# Autodesk Inventor assembly: RR-PCSS-2021-3M1
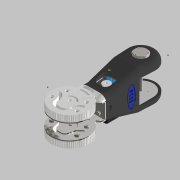
[picture p0: Inventor's stored thumbnail of the model, 180x180]
Saved by Autodesk Inventor 2021 (Build 250183000, 183)
## iProperties
Created: 2021-10-25
Part Number: RR-PCSS-2021-3M1
Document SubType Name: Assembly
Designer: marci
Mass: 2425.99 g
Surface Area: 3551.52 cm^2
Volume: 1267.26 cm^3
Density: 1.91436 g/cm^3
Author: marci
## Documents named in this file (25)
- C:\Users\marci\Desktop\Projekt ramienia\3M1D\RR-PCSS-2021-3M1.iam
- C:\Users\marci\Desktop\Projekt ramienia\3M1D\RR-PCSS-2021-3M1D.ipt
- C:\Users\marci\Desktop\Projekt ramienia\3M1D\RR-PCSS-2021-W3M1.1.ipt
- C:\Users\marci\Desktop\Projekt ramienia\3M1D\RR-PCSS-2021-MSK.ipt
- C:\Users\marci\Desktop\Projekt ramienia\3M1D\Nema 17 Reductor.ipt
- C:\Users\marci\Desktop\Projekt ramienia\3M1D\Pulley 8mm IGNIS.ipt
- C:\Users\marci\Desktop\Projekt ramienia\2M2\RR-PCSS-2021-W2M2MA.ipt
- C:\Users\marci\Desktop\Projekt ramienia\Nowy folder\pl-PL\ISO 4762(2)\ISO 4762 - M6 x 12ISO.ipt
- C:\Users\marci\Desktop\Projekt ramienia\Nowy folder\pl-PL\ISO 7089\ISO 7089 - 6 - 140 HV(1).ipt
- C:\Users\marci\Desktop\Projekt ramienia\Nowy folder\pl-PL\ISO 4035(2)\ISO 4035 - M6 - ISO.ipt
- C:\Users\marci\Desktop\Projekt ramienia\2M2\RR-PCSS-2021-2M2.ipt
- C:\Users\marci\Desktop\Projekt ramienia\Nowy folder\pl-PL\ANSI B18.3.1M(6)\ANSI B18.3.1M - M3x0,5 x 45(1).ipt
- C:\Users\marci\Desktop\Projekt ramienia\Nowy folder\pl-PL\ISO 7092\ISO 7092 - ST 3 - 140 HV.ipt
- C:\Users\marci\Desktop\Projekt ramienia\Nowy folder\pl-PL\ISO 4036(2)\ISO 4036 - M3(2).ipt
- C:\Users\marci\Desktop\Projekt ramienia\3M1D\Tapa 3M1C.ipt
- C:\Users\marci\Desktop\Projekt ramienia\3M1D\T3M1.iam
- C:\Users\marci\Desktop\Projekt ramienia\Nowy folder\pl-PL\ISO 4762(2)\ISO 4762 - M4 x 6ISO.ipt
- C:\Users\marci\Desktop\Projekt ramienia\Nowy folder\pl-PL\ISO 4762(2)\ISO 4762 - M3 x 25ISO.ipt
- C:\Users\marci\Desktop\Projekt ramienia\Nowy folder\pl-PL\ISO 4762(2)\ISO 4762 - M5 x 16ISO.ipt
- C:\Users\marci\Desktop\Projekt ramienia\Nowy folder\pl-PL\ISO 4762(2)\ISO 4762 - M3 x 6ISO.ipt
- C:\Users\marci\Desktop\Projekt ramienia\3M1D\8mm Bearing.ipt
- C:\Users\marci\Desktop\Projekt ramienia\Nowy folder\pl-PL\ISO 4161\ISO 4161 - M8(1).ipt
- C:\Users\marci\Desktop\Projekt ramienia\Nowy folder\pl-PL\ISO 4762(2)\ISO 4762 - M6 x 20ISO.ipt
- C:\Users\marci\Desktop\Projekt ramienia\Nowy folder\pl-PL\ISO 4161\ISO 4161 - M6(1).ipt
- C:\Users\marci\Desktop\Projekt ramienia\Nowy folder\pl-PL\AS 1111\AS 1111 - M8 x 120.ipt
## Components (59 placed, 24 different names)
1. RR-PCSS-2021-W3M1.1:1 — Wstawiające:1, Zestawiające:1, Równoległe:1, Zestawiające:2, Zestawiające:8, Zestawiające:9, Zestawiające:11, Zestawiające:12, Zestawiające:13, Zestawiające:14, Zestawiające:15, Zestawiające:16, Zestawiające:17, Zestawiające:18, Zestawiające:19, Zestawiające:21, Zestawiające:23, Zestawiające:25
2. RR-PCSS-2021-3M1D:1 — Wstawiające:1, Zestawiające:27, Zestawiające:28, Zestawiające:29, Zestawiające:30, Zestawiające:31, Zestawiające:33, Zestawiające:34, Zestawiające:35, Zestawiające:36, Zestawiające:37, Zestawiające:50, Zestawiające:51, Zestawiające:52, Wstawiające:11, Wstawiające:12
3. RR-PCSS-2021-MSK:1 — Zestawiające:1, Równoległe:1, Zestawiające:2, Wstawiające:2, Zestawiające:32, Zestawiające:39, Zestawiające:40, Zestawiające:41, Zestawiające:42, Zestawiające:43, Zestawiające:53, Zestawiające:54, Zestawiające:55, Zestawiające:56, Zestawiające:57, Zestawiające:58, Zestawiające:59, Zestawiające:60
4. Nema 17 Reductor:1 — Wstawiające:2, Wstawiające:3, Zestawiające:10
5. Pulley 8mm IGNIS:1 — Wstawiające:3
6. RR-PCSS-2021-W2M2MA:1 — Zestawiające:8, Zestawiające:9, Zestawiające:10, Zestawiające:20, Zestawiające:22, Zestawiające:24, Zestawiające:26, Wstawiające:8, Wstawiające:9, Zestawiające:80, Zestawiające:82, Zestawiające:84, Zestawiające:86, Zestawiające:96, Zestawiające:98, Zestawiające:100, Zestawiające:102
7. ISO 4762 M6 x 12:1 — Zestawiające:11, Zestawiające:12
8. ISO 7089 6:1 — Zestawiające:19, Zestawiające:20, Wstawiające:4
9. ISO 4035 M6:1 — Wstawiające:4
10. ISO 4762 M6 x 12:2 — Zestawiające:13, Zestawiające:14
11. ISO 4762 M6 x 12:3 — Zestawiające:15, Zestawiające:16
12. ISO 4762 M6 x 12:4 — Zestawiające:17, Zestawiające:18
13. ISO 7089 6:2 — Zestawiające:21, Zestawiające:22, Wstawiające:5
14. ISO 7089 6:3 — Zestawiające:23, Zestawiające:24, Wstawiające:6
15. ISO 7089 6:4 — Zestawiające:25, Zestawiające:26, Wstawiające:7
16. ISO 4035 M6:2 — Wstawiające:5
17. ISO 4035 M6:3 — Wstawiające:6
18. ISO 4035 M6:4 — Wstawiające:7
19. RR-PCSS-2021-2M2:1 — Wstawiające:9, Zestawiające:28, Zestawiające:71, Zestawiające:72, Zestawiające:73, Zestawiające:74, Zestawiające:75, Zestawiające:76, Zestawiające:77, Zestawiające:78, Zestawiające:79, Zestawiające:81, Zestawiające:83, Zestawiające:85
20. RR-PCSS-2021-2M2:2 — Wstawiające:8, Zestawiające:27, Zestawiające:87, Zestawiające:88, Zestawiające:89, Zestawiające:90, Zestawiające:91, Zestawiające:92, Zestawiające:93, Zestawiające:94, Zestawiające:95, Zestawiające:97, Zestawiające:99, Zestawiające:101
21. Wkręt z łbem o zmniejszonych wymiarach z gniazdem kutym - Metryczny M3x0,5 x 45:1 — Zestawiające:29, Zestawiające:30, Zestawiające:38
22. ISO 7092 ST 3 - 140 HV:1 — Zestawiające:31, Zestawiające:32, Wstawiające:10
23. ISO 4036 M3:1 — Wstawiające:10
24. Tapa 3M1C:1 — Zestawiające:33, Zestawiające:34, Zestawiające:35, Zestawiające:107, Zestawiające:108, Zestawiające:109, Zestawiające:110, Zestawiające:111, Zestawiające:112
25. Tapa 3M1C:2 — Zestawiające:36, Zestawiające:37, Zestawiające:44, Zestawiające:45, Zestawiające:46, Zestawiające:47, Zestawiające:48, Zestawiające:49
26. T3M1:1 [sub-assembly] — Zestawiające:38, Zestawiające:39
27. ISO 4762 M4 x 6:1 — Zestawiające:40, Zestawiające:41
28. ISO 4762 M4 x 6:2 — Zestawiające:42, Zestawiające:43
29. ISO 4762 M3 x 25:1 — Zestawiające:44, Zestawiające:45
30. ISO 4762 M3 x 25:2 — Zestawiające:46, Zestawiające:47, Zestawiające:50
31. ISO 4762 M3 x 25:3 — Zestawiające:48, Zestawiające:49
32. ISO 4762 M5 x 16:1 — Zestawiające:51, Zestawiające:52
33. ISO 4762 M3 x 6:1 — Zestawiające:53, Zestawiające:54
34. ISO 4762 M3 x 6:2 — Zestawiające:55, Zestawiające:56
35. ISO 4762 M3 x 6:3 — Zestawiające:57, Zestawiające:58
36. ISO 4762 M3 x 6:4 — Zestawiające:59, Zestawiające:60
37. ISO 4762 M3 x 25:4 — Zestawiające:107, Zestawiające:108
38. 8mm Bearing:1 — Wstawiające:12, Zestawiające:106
39. 8mm Bearing:2 — Wstawiające:11, Zestawiające:103, Zestawiające:104, Zestawiające:105
40. AS 1111 - Metryczny M8 x 120:1 — Zestawiające:103, Zestawiające:104
41. ISO 4161 M8:1 — Zestawiające:105, Zestawiające:106
42. ISO 4762 M6 x 20:1 — Zestawiające:71, Zestawiające:72
43. ISO 4161 M6:1 — Zestawiające:79, Zestawiające:80
44. ISO 4762 M6 x 20:2 — Zestawiające:73, Zestawiające:74
45. ISO 4762 M6 x 20:3 — Zestawiające:75, Zestawiające:76
46. ISO 4762 M6 x 20:4 — Zestawiające:77, Zestawiające:78
47. ISO 4161 M6:2 — Zestawiające:81, Zestawiające:82
48. ISO 4161 M6:3 — Zestawiające:83, Zestawiające:84
49. ISO 4161 M6:4 — Zestawiające:85, Zestawiające:86
50. ISO 4762 M6 x 20:5 — Zestawiające:87, Zestawiające:88
51. ISO 4161 M6:5 — Zestawiające:95, Zestawiające:96
52. ISO 4762 M6 x 20:6 — Zestawiające:89, Zestawiające:90
53. ISO 4762 M6 x 20:7 — Zestawiające:91, Zestawiające:92
54. ISO 4762 M6 x 20:8 — Zestawiające:93, Zestawiające:94
55. ISO 4161 M6:6 — Zestawiające:97, Zestawiające:98
56. ISO 4161 M6:7 — Zestawiające:99, Zestawiające:100
57. ISO 4161 M6:8 — Zestawiające:101, Zestawiające:102
58. ISO 4762 M3 x 25:5 — Zestawiające:109, Zestawiające:110
59. ISO 4762 M3 x 25:6 — Zestawiające:111, Zestawiające:112
## Relationships (110: Mate 97, Insert 12, Flush 1)
- Wstawiające:1 [Insert]: RR-PCSS-2021-W3M1.1:1 ↔ RR-PCSS-2021-3M1D:1
- Zestawiające:1 [Mate]: RR-PCSS-2021-W3M1.1:1 ↔ RR-PCSS-2021-MSK:1
- Równoległe:1 [Flush] (-50 mm): RR-PCSS-2021-W3M1.1:1 ↔ RR-PCSS-2021-MSK:1
- Zestawiające:2 [Mate] (3 mm): RR-PCSS-2021-W3M1.1:1 ↔ RR-PCSS-2021-MSK:1
- Wstawiające:2 [Insert]: RR-PCSS-2021-MSK:1 ↔ Nema 17 Reductor:1
- Wstawiające:3 [Insert]: Nema 17 Reductor:1 ↔ Pulley 8mm IGNIS:1
- Zestawiające:8 [Mate]: RR-PCSS-2021-W3M1.1:1 ↔ RR-PCSS-2021-W2M2MA:1
- Zestawiające:9 [Mate] (13 mm): RR-PCSS-2021-W3M1.1:1 ↔ RR-PCSS-2021-W2M2MA:1
- Zestawiające:10 [Mate] (19.035 mm): Nema 17 Reductor:1 ↔ RR-PCSS-2021-W2M2MA:1
- Zestawiające:11 [Mate]: RR-PCSS-2021-W3M1.1:1 ↔ ISO 4762 M6 x 12:1
- Zestawiające:12 [Mate]: RR-PCSS-2021-W3M1.1:1 ↔ ISO 4762 M6 x 12:1
- Zestawiające:13 [Mate]: RR-PCSS-2021-W3M1.1:1 ↔ ISO 4762 M6 x 12:2
- Zestawiające:14 [Mate]: RR-PCSS-2021-W3M1.1:1 ↔ ISO 4762 M6 x 12:2
- Zestawiające:15 [Mate]: RR-PCSS-2021-W3M1.1:1 ↔ ISO 4762 M6 x 12:3
- Zestawiające:16 [Mate]: RR-PCSS-2021-W3M1.1:1 ↔ ISO 4762 M6 x 12:3
- Zestawiające:17 [Mate]: RR-PCSS-2021-W3M1.1:1 ↔ ISO 4762 M6 x 12:4
- Zestawiające:18 [Mate]: RR-PCSS-2021-W3M1.1:1 ↔ ISO 4762 M6 x 12:4
- Zestawiające:19 [Mate]: RR-PCSS-2021-W3M1.1:1 ↔ ISO 7089 6:1
- Zestawiające:20 [Mate]: RR-PCSS-2021-W2M2MA:1 ↔ ISO 7089 6:1
- Zestawiające:21 [Mate]: RR-PCSS-2021-W3M1.1:1 ↔ ISO 7089 6:2
- Zestawiające:22 [Mate]: RR-PCSS-2021-W2M2MA:1 ↔ ISO 7089 6:2
- Zestawiające:23 [Mate]: RR-PCSS-2021-W3M1.1:1 ↔ ISO 7089 6:3
- Zestawiające:24 [Mate]: RR-PCSS-2021-W2M2MA:1 ↔ ISO 7089 6:3
- Zestawiające:25 [Mate]: RR-PCSS-2021-W3M1.1:1 ↔ ISO 7089 6:4
- Zestawiające:26 [Mate]: RR-PCSS-2021-W2M2MA:1 ↔ ISO 7089 6:4
- Wstawiające:4 [Insert]: ISO 7089 6:1 ↔ ISO 4035 M6:1
- Wstawiające:5 [Insert]: ISO 7089 6:2 ↔ ISO 4035 M6:2
- Wstawiające:6 [Insert]: ISO 7089 6:3 ↔ ISO 4035 M6:3
- Wstawiające:7 [Insert]: ISO 7089 6:4 ↔ ISO 4035 M6:4
- Wstawiające:8 [Insert]: RR-PCSS-2021-W2M2MA:1 ↔ RR-PCSS-2021-2M2:2
- Zestawiające:27 [Mate]: RR-PCSS-2021-3M1D:1 ↔ RR-PCSS-2021-2M2:2
- Wstawiające:9 [Insert]: RR-PCSS-2021-W2M2MA:1 ↔ RR-PCSS-2021-2M2:1
- Zestawiające:28 [Mate]: RR-PCSS-2021-3M1D:1 ↔ RR-PCSS-2021-2M2:1
- Zestawiające:29 [Mate]: RR-PCSS-2021-3M1D:1 ↔ Wkręt z łbem o zmniejszonych wymiarach z gniazdem kutym - Metryczny M3x0,5 x 45:1
- Zestawiające:30 [Mate]: RR-PCSS-2021-3M1D:1 ↔ Wkręt z łbem o zmniejszonych wymiarach z gniazdem kutym - Metryczny M3x0,5 x 45:1
- Zestawiające:31 [Mate]: RR-PCSS-2021-3M1D:1 ↔ ISO 7092 ST 3 - 140 HV:1
- Zestawiające:32 [Mate]: RR-PCSS-2021-MSK:1 ↔ ISO 7092 ST 3 - 140 HV:1
- Wstawiające:10 [Insert]: ISO 7092 ST 3 - 140 HV:1 ↔ ISO 4036 M3:1
- Zestawiające:33 [Mate]: RR-PCSS-2021-3M1D:1 ↔ Tapa 3M1C:1
- Zestawiające:34 [Mate]: RR-PCSS-2021-3M1D:1 ↔ Tapa 3M1C:1
- Zestawiające:35 [Mate]: RR-PCSS-2021-3M1D:1 ↔ Tapa 3M1C:1
- Zestawiające:36 [Mate]: RR-PCSS-2021-3M1D:1 ↔ Tapa 3M1C:2
- Zestawiające:37 [Mate]: RR-PCSS-2021-3M1D:1 ↔ Tapa 3M1C:2
- Zestawiające:38 [Mate]: Wkręt z łbem o zmniejszonych wymiarach z gniazdem kutym - Metryczny M3x0,5 x 45:1 ↔ T3M1:1
- Zestawiające:39 [Mate] (2 mm): RR-PCSS-2021-MSK:1 ↔ T3M1:1
- Zestawiające:40 [Mate]: RR-PCSS-2021-MSK:1 ↔ ISO 4762 M4 x 6:1
- Zestawiające:41 [Mate]: RR-PCSS-2021-MSK:1 ↔ ISO 4762 M4 x 6:1
- Zestawiające:42 [Mate]: RR-PCSS-2021-MSK:1 ↔ ISO 4762 M4 x 6:2
- Zestawiające:43 [Mate]: RR-PCSS-2021-MSK:1 ↔ ISO 4762 M4 x 6:2
- Zestawiające:44 [Mate]: Tapa 3M1C:2 ↔ ISO 4762 M3 x 25:1
- Zestawiające:45 [Mate]: Tapa 3M1C:2 ↔ ISO 4762 M3 x 25:1
- Zestawiające:46 [Mate]: Tapa 3M1C:2 ↔ ISO 4762 M3 x 25:2
- Zestawiające:47 [Mate]: Tapa 3M1C:2 ↔ ISO 4762 M3 x 25:2
- Zestawiające:48 [Mate]: Tapa 3M1C:2 ↔ ISO 4762 M3 x 25:3
- Zestawiające:49 [Mate]: Tapa 3M1C:2 ↔ ISO 4762 M3 x 25:3
- Zestawiające:50 [Mate]: RR-PCSS-2021-3M1D:1 ↔ ISO 4762 M3 x 25:2
- Zestawiające:51 [Mate]: RR-PCSS-2021-3M1D:1 ↔ ISO 4762 M5 x 16:1
- Zestawiające:52 [Mate]: RR-PCSS-2021-3M1D:1 ↔ ISO 4762 M5 x 16:1
- Zestawiające:53 [Mate]: RR-PCSS-2021-MSK:1 ↔ ISO 4762 M3 x 6:1
- Zestawiające:54 [Mate]: RR-PCSS-2021-MSK:1 ↔ ISO 4762 M3 x 6:1
- Zestawiające:55 [Mate]: RR-PCSS-2021-MSK:1 ↔ ISO 4762 M3 x 6:2
- Zestawiające:56 [Mate]: RR-PCSS-2021-MSK:1 ↔ ISO 4762 M3 x 6:2
- Zestawiające:57 [Mate]: RR-PCSS-2021-MSK:1 ↔ ISO 4762 M3 x 6:3
- Zestawiające:58 [Mate]: RR-PCSS-2021-MSK:1 ↔ ISO 4762 M3 x 6:3
- Zestawiające:59 [Mate]: RR-PCSS-2021-MSK:1 ↔ ISO 4762 M3 x 6:4
- Zestawiające:60 [Mate]: RR-PCSS-2021-MSK:1 ↔ ISO 4762 M3 x 6:4
- Wstawiające:11 [Insert]: RR-PCSS-2021-3M1D:1 ↔ 8mm Bearing:2
- Wstawiające:12 [Insert]: RR-PCSS-2021-3M1D:1 ↔ 8mm Bearing:1
- Zestawiające:71 [Mate]: RR-PCSS-2021-2M2:1 ↔ ISO 4762 M6 x 20:1
- Zestawiające:72 [Mate]: RR-PCSS-2021-2M2:1 ↔ ISO 4762 M6 x 20:1
- Zestawiające:73 [Mate]: RR-PCSS-2021-2M2:1 ↔ ISO 4762 M6 x 20:2
- Zestawiające:74 [Mate]: RR-PCSS-2021-2M2:1 ↔ ISO 4762 M6 x 20:2
- Zestawiające:75 [Mate]: RR-PCSS-2021-2M2:1 ↔ ISO 4762 M6 x 20:3
- Zestawiające:76 [Mate]: RR-PCSS-2021-2M2:1 ↔ ISO 4762 M6 x 20:3
- Zestawiające:77 [Mate]: RR-PCSS-2021-2M2:1 ↔ ISO 4762 M6 x 20:4
- Zestawiające:78 [Mate]: RR-PCSS-2021-2M2:1 ↔ ISO 4762 M6 x 20:4
- Zestawiające:79 [Mate]: RR-PCSS-2021-2M2:1 ↔ ISO 4161 M6:1
- Zestawiające:80 [Mate]: RR-PCSS-2021-W2M2MA:1 ↔ ISO 4161 M6:1
- Zestawiające:81 [Mate]: RR-PCSS-2021-2M2:1 ↔ ISO 4161 M6:2
- Zestawiające:82 [Mate]: RR-PCSS-2021-W2M2MA:1 ↔ ISO 4161 M6:2
- Zestawiające:83 [Mate]: RR-PCSS-2021-2M2:1 ↔ ISO 4161 M6:3
- Zestawiające:84 [Mate]: RR-PCSS-2021-W2M2MA:1 ↔ ISO 4161 M6:3
- Zestawiające:85 [Mate]: RR-PCSS-2021-2M2:1 ↔ ISO 4161 M6:4
- Zestawiające:86 [Mate]: RR-PCSS-2021-W2M2MA:1 ↔ ISO 4161 M6:4
- Zestawiające:87 [Mate]: RR-PCSS-2021-2M2:2 ↔ ISO 4762 M6 x 20:5
- Zestawiające:88 [Mate]: RR-PCSS-2021-2M2:2 ↔ ISO 4762 M6 x 20:5
- Zestawiające:89 [Mate]: RR-PCSS-2021-2M2:2 ↔ ISO 4762 M6 x 20:6
- Zestawiające:90 [Mate]: RR-PCSS-2021-2M2:2 ↔ ISO 4762 M6 x 20:6
- Zestawiające:91 [Mate]: RR-PCSS-2021-2M2:2 ↔ ISO 4762 M6 x 20:7
- Zestawiające:92 [Mate]: RR-PCSS-2021-2M2:2 ↔ ISO 4762 M6 x 20:7
- Zestawiające:93 [Mate]: RR-PCSS-2021-2M2:2 ↔ ISO 4762 M6 x 20:8
- Zestawiające:94 [Mate]: RR-PCSS-2021-2M2:2 ↔ ISO 4762 M6 x 20:8
- Zestawiające:95 [Mate]: RR-PCSS-2021-2M2:2 ↔ ISO 4161 M6:5
- Zestawiające:96 [Mate]: RR-PCSS-2021-W2M2MA:1 ↔ ISO 4161 M6:5
- Zestawiające:97 [Mate]: RR-PCSS-2021-2M2:2 ↔ ISO 4161 M6:6
- Zestawiające:98 [Mate]: RR-PCSS-2021-W2M2MA:1 ↔ ISO 4161 M6:6
- Zestawiające:99 [Mate]: RR-PCSS-2021-2M2:2 ↔ ISO 4161 M6:7
- Zestawiające:100 [Mate]: RR-PCSS-2021-W2M2MA:1 ↔ ISO 4161 M6:7
- Zestawiające:101 [Mate]: RR-PCSS-2021-2M2:2 ↔ ISO 4161 M6:8
- Zestawiające:102 [Mate]: RR-PCSS-2021-W2M2MA:1 ↔ ISO 4161 M6:8
- Zestawiające:103 [Mate]: 8mm Bearing:2 ↔ AS 1111 - Metryczny M8 x 120:1
- Zestawiające:104 [Mate]: 8mm Bearing:2 ↔ AS 1111 - Metryczny M8 x 120:1
- Zestawiające:105 [Mate]: 8mm Bearing:2 ↔ ISO 4161 M8:1
- Zestawiające:106 [Mate]: 8mm Bearing:1 ↔ ISO 4161 M8:1
- Zestawiające:107 [Mate]: Tapa 3M1C:1 ↔ ISO 4762 M3 x 25:4
- Zestawiające:108 [Mate]: Tapa 3M1C:1 ↔ ISO 4762 M3 x 25:4
- Zestawiające:109 [Mate]: Tapa 3M1C:1 ↔ ISO 4762 M3 x 25:5
- Zestawiające:110 [Mate]: Tapa 3M1C:1 ↔ ISO 4762 M3 x 25:5
- Zestawiające:111 [Mate]: Tapa 3M1C:1 ↔ ISO 4762 M3 x 25:6
- Zestawiające:112 [Mate]: Tapa 3M1C:1 ↔ ISO 4762 M3 x 25:6
